# Autodesk Inventor assembly: Bend Piece 1764
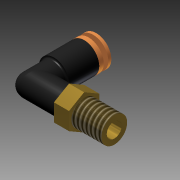
[picture p0: Inventor's stored thumbnail of the model, 180x180]
Saved by Autodesk Inventor 2011 (Build 150239000, 239)
## iProperties
Created: 2010-02-15
Part Number: Bend Piece 1764
Document SubType Name: Assembly
Designer: jgehrig
Author: jgehrig
## Documents named in this file (4)
- R:\CAD Archives\Pneumatics\Regulator 1764\Pnewmatics Bend Piece 1764\Pneumatic Bend Piece 1764.iam
- R:\CAD Archives\Pneumatics\Regulator 1764\Pnewmatics Bend Piece 1764\Pneumatic Bend Piece 1764.ipt
- R:\CAD Archives\Pneumatics\Regulator 1764\Pnewmatics Bend Piece 1764\Pneumatic Screw Part 1764.ipt
- R:\CAD Archives\Pneumatics\Regulator 1764\Pnewmatics Bend Piece 1764\Pneumatic Screw Part 2 1764.ipt
## Components (3 placed, 3 different names)
1. Pneumatic Bend Piece 1764:1 — Insert:1, Insert:2
2. Pneumatic Screw Part 1764:1 — Insert:2
3. Pneumatic Screw Part 2 1764:1 — Insert:1
## Relationships (2: Insert 2)
- Insert:1: Pneumatic Bend Piece 1764:1 ↔ Pneumatic Screw Part 2 1764:1
- Insert:2: Pneumatic Bend Piece 1764:1 ↔ Pneumatic Screw Part 1764:1
